# Autodesk Inventor assembly: Сборка1
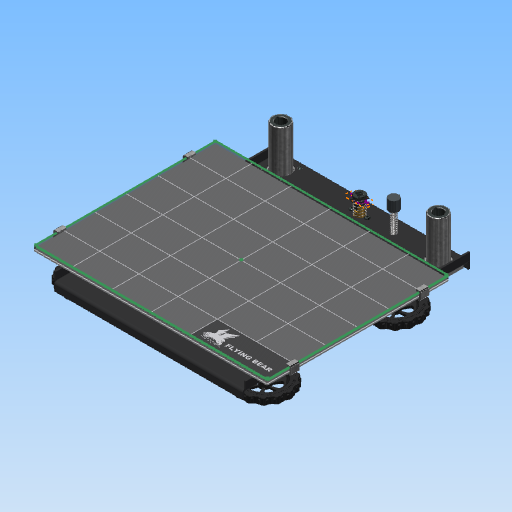
[picture p0: Inventor's stored thumbnail of the model, 512x512]
Saved by Autodesk Inventor 2017 (Build 210142000, 142)
## iProperties
Part Number: Сборка1
Material: Типовые
Document SubType Name: Assembly
Designer: Max
Author: Max
## Documents named in this file (15)
- C:\Users\Max\Desktop\Flying Bear Ghost 5\table assembly.iam
- C:\Users\Max\Desktop\Flying Bear Ghost 5\screw m3.ipt
- C:\Users\Max\Desktop\Flying Bear Ghost 5\Bed level springs.ipt
- C:\Users\Max\Desktop\Flying Bear Ghost 5\LMK12LUU.ipt
- C:\Users\Max\Desktop\Flying Bear Ghost 5\z-nut screw t8.ipt
- C:\Users\Max\Desktop\Flying Bear Ghost 5\Hand Twisted Nut.ipt
- C:\Users\Max\Desktop\Flying Bear Ghost 5\z-nut screw t8 2.ipt
- C:\Users\Max\Desktop\Flying Bear Ghost 5\spring t8.ipt
- C:\Users\Max\Desktop\Flying Bear Ghost 5\table frame.ipt
- C:\Users\Max\Desktop\Flying Bear Ghost 5\table.ipt
- C:\Users\Max\Desktop\Flying Bear Ghost 5\ultrabase.ipt
- C:\Users\Max\Desktop\Flying Bear Ghost 5\limit switch adjusting screw.ipt
- C:\Users\Max\Desktop\Flying Bear Ghost 5\limit switch spring.ipt
- C:\Users\Max\Desktop\Flying Bear Ghost 5\staple.ipt
- C:\Users\Max\Desktop\Flying Bear Ghost 5\factory table insulation.ipt
## Components (33 placed, 14 different names)
1. Bed level springs:1 — Заподлицо:81, Совмещение:205, Совмещение:206
2. LMK12LUU:1 — Заподлицо:58, Заподлицо:59, Заподлицо:67, Совмещение:178, Совмещение:189, Совмещение:190, Совмещение:191, Совмещение:192, Совмещение:193
3. z-nut screw t8:1 — Заподлицо:67, Совмещение:170, Совмещение:171, Совмещение:173
4. Hand Twisted Nut:1 — Совмещение:196, Заподлицо:78, Совмещение:200
5. LMK12LUU:2 — Заподлицо:58, Заподлицо:59, Совмещение:179, Совмещение:180, Совмещение:184, Совмещение:185, Совмещение:186, Совмещение:187, Совмещение:188
6. z-nut screw t8 2:1 — Совмещение:170, Совмещение:171
7. spring t8:1 — Совмещение:173
8. table frame:1 — Совмещение:178, Совмещение:179, Совмещение:180, Совмещение:181, Совмещение:182, Совмещение:183, Совмещение:194, Совмещение:195, Совмещение:200, Совмещение:201, Совмещение:206, Совмещение:255, Совмещение:256, Совмещение:258
9. screw m3:19 — Совмещение:182, Заподлицо:69, Совмещение:183
10. screw m3:20 — Совмещение:181, Заподлицо:69
11. screw m3:21 — Заподлицо:70, Совмещение:184
12. screw m3:22 — Заподлицо:70, Заподлицо:71, Совмещение:185, Совмещение:188
13. screw m3:23 — Заподлицо:72, Совмещение:186
14. screw m3:24 — Заподлицо:71, Заподлицо:72, Совмещение:187
15. screw m3:25 — Совмещение:190, Совмещение:193
16. screw m3:26 — Совмещение:191
17. screw m3:27 — Совмещение:189
18. screw m3:28 — Совмещение:192
19. table:2 — Совмещение:194, Совмещение:195, Совмещение:196, Совмещение:197, Совмещение:198, Совмещение:199, Совмещение:201, Совмещение:202, Совмещение:203, Совмещение:204, Совмещение:205, Заподлицо:82, Заподлицо:83, Заподлицо:84, Совмещение:262, Заподлицо:101, Совмещение:263, Совмещение:435, Заподлицо:161, Заподлицо:162
20. Hand Twisted Nut:2 — Совмещение:197, Заподлицо:76, Заподлицо:77
21. Hand Twisted Nut:3 — Совмещение:198, Заподлицо:76
22. Hand Twisted Nut:4 — Совмещение:199, Заподлицо:77, Заподлицо:78
23. Bed level springs:2 — Заподлицо:80, Заподлицо:81, Совмещение:204
24. Bed level springs:3 — Заподлицо:79, Заподлицо:80, Совмещение:202
25. Bed level springs:4 — Заподлицо:79, Совмещение:203
26. ultrabase:1 — Заподлицо:82, Заподлицо:83, Заподлицо:84, Совмещение:261, Заподлицо:102
27. limit switch adjusting screw:1 — Совмещение:255, Совмещение:256, Совмещение:257
28. limit switch spring:1 — Совмещение:257, Совмещение:258
29. staple:1 — Совмещение:261, Совмещение:262, Заподлицо:99, Заподлицо:100, Заподлицо:101, Заподлицо:105, Заподлицо:106
30. staple:2 — Заподлицо:99, Заподлицо:100, Заподлицо:102, Заподлицо:107
31. staple:3 — Заподлицо:103, Заподлицо:104, Совмещение:263, Заподлицо:106
32. staple:4 — Заподлицо:103, Заподлицо:104, Заподлицо:105, Заподлицо:107
33. factory table insulation:1 — Совмещение:435, Заподлицо:161, Заподлицо:162
## Relationships (70: Mate 40, Flush 30)
- Заподлицо:58 [Flush]: LMK12LUU:1 ↔ LMK12LUU:2
- Заподлицо:59 [Flush]: LMK12LUU:1 ↔ LMK12LUU:2
- Заподлицо:67 [Flush]: LMK12LUU:1 ↔ z-nut screw t8:1
- Совмещение:170 [Mate]: z-nut screw t8:1 ↔ z-nut screw t8 2:1
- Совмещение:171 [Mate] (1 mm): z-nut screw t8:1 ↔ z-nut screw t8 2:1
- Совмещение:173 [Mate]: z-nut screw t8:1 ↔ spring t8:1
- Совмещение:178 [Mate]: LMK12LUU:1 ↔ table frame:1
- Совмещение:179 [Mate]: LMK12LUU:2 ↔ table frame:1
- Совмещение:180 [Mate]: LMK12LUU:2 ↔ table frame:1
- Совмещение:181 [Mate]: table frame:1 ↔ screw m3:20
- Совмещение:182 [Mate]: table frame:1 ↔ screw m3:19
- Заподлицо:69 [Flush]: screw m3:19 ↔ screw m3:20
- Совмещение:183 [Mate]: table frame:1 ↔ screw m3:19
- Заподлицо:70 [Flush]: screw m3:21 ↔ screw m3:22
- Заподлицо:71 [Flush]: screw m3:22 ↔ screw m3:24
- Заподлицо:72 [Flush]: screw m3:23 ↔ screw m3:24
- Совмещение:184 [Mate]: LMK12LUU:2 ↔ screw m3:21
- Совмещение:185 [Mate]: LMK12LUU:2 ↔ screw m3:22
- Совмещение:186 [Mate]: LMK12LUU:2 ↔ screw m3:23
- Совмещение:187 [Mate]: LMK12LUU:2 ↔ screw m3:24
- [Flush]: screw m3:25 ↔ screw m3:26
- [Flush]: screw m3:26 ↔ screw m3:28
- [Flush]: screw m3:27 ↔ screw m3:28
- Совмещение:188 [Mate]: LMK12LUU:2 ↔ screw m3:22
- Совмещение:189 [Mate]: LMK12LUU:1 ↔ screw m3:27
- Совмещение:190 [Mate]: LMK12LUU:1 ↔ screw m3:25
- Совмещение:191 [Mate]: LMK12LUU:1 ↔ screw m3:26
- Совмещение:192 [Mate]: LMK12LUU:1 ↔ screw m3:28
- Совмещение:193 [Mate]: LMK12LUU:1 ↔ screw m3:25
- Совмещение:194 [Mate]: table frame:1 ↔ table:2
- Совмещение:195 [Mate]: table frame:1 ↔ table:2
- Совмещение:196 [Mate]: Hand Twisted Nut:1 ↔ table:2
- Совмещение:197 [Mate]: table:2 ↔ Hand Twisted Nut:2
- Совмещение:198 [Mate]: table:2 ↔ Hand Twisted Nut:3
- Совмещение:199 [Mate]: table:2 ↔ Hand Twisted Nut:4
- Заподлицо:76 [Flush]: Hand Twisted Nut:2 ↔ Hand Twisted Nut:3
- Заподлицо:77 [Flush]: Hand Twisted Nut:2 ↔ Hand Twisted Nut:4
- Заподлицо:78 [Flush]: Hand Twisted Nut:1 ↔ Hand Twisted Nut:4
- Совмещение:200 [Mate]: Hand Twisted Nut:1 ↔ table frame:1
- Совмещение:201 [Mate] (17 mm): table frame:1 ↔ table:2
- Заподлицо:79 [Flush]: Bed level springs:3 ↔ Bed level springs:4
- Заподлицо:80 [Flush]: Bed level springs:2 ↔ Bed level springs:3
- Заподлицо:81 [Flush]: Bed level springs:1 ↔ Bed level springs:2
- Совмещение:202 [Mate]: table:2 ↔ Bed level springs:3
- Совмещение:203 [Mate]: table:2 ↔ Bed level springs:4
- Совмещение:204 [Mate]: table:2 ↔ Bed level springs:2
- Совмещение:205 [Mate]: Bed level springs:1 ↔ table:2
- Совмещение:206 [Mate]: Bed level springs:1 ↔ table frame:1
- Заподлицо:82 [Flush]: table:2 ↔ ultrabase:1
- Заподлицо:83 [Flush]: table:2 ↔ ultrabase:1
- Заподлицо:84 [Flush]: table:2 ↔ ultrabase:1
- Совмещение:255 [Mate]: table frame:1 ↔ limit switch adjusting screw:1
- Совмещение:256 [Mate] (25 mm): table frame:1 ↔ limit switch adjusting screw:1
- Совмещение:257 [Mate]: limit switch adjusting screw:1 ↔ limit switch spring:1
- Совмещение:258 [Mate]: table frame:1 ↔ limit switch spring:1
- Совмещение:261 [Mate]: ultrabase:1 ↔ staple:1
- Совмещение:262 [Mate]: table:2 ↔ staple:1
- Заподлицо:99 [Flush]: staple:1 ↔ staple:2
- Заподлицо:100 [Flush]: staple:1 ↔ staple:2
- Заподлицо:101 [Flush] (26 mm): table:2 ↔ staple:1
- Заподлицо:102 [Flush] (26 mm): ultrabase:1 ↔ staple:2
- Заподлицо:103 [Flush]: staple:3 ↔ staple:4
- Заподлицо:104 [Flush]: staple:3 ↔ staple:4
- Совмещение:263 [Mate]: table:2 ↔ staple:3
- Заподлицо:105 [Flush]: staple:1 ↔ staple:4
- Заподлицо:106 [Flush]: staple:1 ↔ staple:3
- Заподлицо:107 [Flush]: staple:2 ↔ staple:4
- Совмещение:435 [Mate]: table:2 ↔ factory table insulation:1
- Заподлицо:161 [Flush] (20 mm): table:2 ↔ factory table insulation:1
- Заподлицо:162 [Flush] (40 mm): table:2 ↔ factory table insulation:1
## Named parameters: d278_d273 = 0 mm, d279_d271 = 0 mm, d280_d272 = 0 mm
